# Autodesk Inventor assembly: LoadCellA
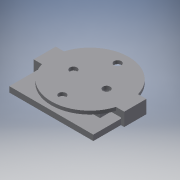
[picture p0: Inventor's stored thumbnail of the model, 180x180]
Saved by Autodesk Inventor 2018 (Build 220112000, 112)
## iProperties
Created: 2018-05-09
Part Number: LoadCellA
Document SubType Name: Assembly
Designer: s4321966
Author: s4321966
## Documents named in this file (3)
- H:\Inventor-Workspace\METR4901\Load Cell Mount\LoadCellA.iam
- H:\Inventor-Workspace\METR4901\Load Cell Mount\loadCell.ipt
- H:\Inventor-Workspace\METR4901\Load Cell Mount\loadCelMountLower.ipt
## Components (2 placed, 2 different names)
1. loadCell:1 — Flush:1, Mate:1, Mate:2, Flush:2
2. loadCelMountLower:1 — Flush:1, Mate:1, Mate:2, Flush:2
## Relationships (4: Flush 2, Mate 2)
- Flush:1: loadCell:1 ↔ loadCelMountLower:1
- Mate:1: loadCell:1 ↔ loadCelMountLower:1
- Mate:2: loadCell:1 ↔ loadCelMountLower:1
- Flush:2: loadCell:1 ↔ loadCelMountLower:1
